# Autodesk Inventor assembly: コガネイ_BDA16X5
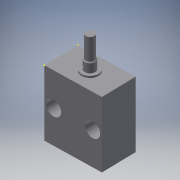
[picture p0: Inventor's stored thumbnail of the model, 180x180]
Saved by Autodesk Inventor 2018 (Build 220112000, 112)
## iProperties
Created: 2018-04-23
Part Number: コガネイ_BDA16X5
Material: 一般
Document SubType Name: Assembly
Designer: Take
Author: Take
## Documents named in this file (3)
- C:\Users\Take\Documents\Inventor\パーツ\コガネイ_BDA16X5.iam
- C:\Users\Take\Documents\Inventor\パーツ\コガネイ_BDA16x5(円柱).ipt
- C:\Users\Take\Documents\Inventor\パーツ\コガネイ_BDA16x5(本体).ipt
## Components (2 placed, 2 different names)
1. コガネイ_BDA16x5(円柱):1 — 円柱状:2
2. コガネイ_BDA16x5(本体):1 — 円柱状:2
## Relationships (1: CylindricalJoint 1)
- 円柱状:2 [CylindricalJoint]: コガネイ_BDA16x5(円柱):1 ↔ コガネイ_BDA16x5(本体):1
